# Autodesk Inventor assembly: HbthumbU02
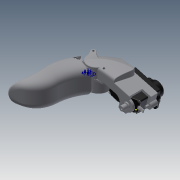
[picture p0: Inventor's stored thumbnail of the model, 180x180]
Saved by Autodesk Inventor 2015 SP1 (Build 190203100, 203)
## iProperties
Created: 2015-02-19
Part Number: HbthumbU02
Document SubType Name: Assembly
Designer: Yamaura
Author: Yamaura
## Documents named in this file (11)
- C:\Users\Yamaura\Documents\GitHub\HACKberry\HACKberry-hardware\3D\Inventor\Parts\HbthumbU02.iam
- C:\Users\Yamaura\Documents\GitHub\HACKberry\HACKberry-hardware\3D\Inventor\Parts\ASV-15MG.ipt
- C:\Users\Yamaura\Documents\GitHub\HACKberry\HACKberry-hardware\3D\Inventor\Parts\HbThumbLockButton01.ipt
- C:\Users\Yamaura\Documents\GitHub\HACKberry\HACKberry-hardware\3D\Inventor\Parts\CP 0.5-6-8.ipt
- C:\Users\Yamaura\Documents\GitHub\HACKberry\HACKberry-hardware\3D\Inventor\Parts\flatScrewM2L6PHI3.3T1.3.ipt
- C:\Users\Yamaura\Documents\GitHub\HACKberry\HACKberry-hardware\3D\Inventor\Parts\ScrewM2L10.ipt
- C:\Users\Yamaura\Documents\GitHub\HACKberry\HACKberry-hardware\3D\Inventor\Parts\HbThumbJointHolder01.ipt
- C:\Users\Yamaura\Documents\GitHub\HACKberry\HACKberry-hardware\3D\Inventor\Parts\HbThumbMetacarpalPhalanx02.ipt
- C:\Users\Yamaura\Documents\GitHub\HACKberry\HACKberry-hardware\3D\Inventor\Parts\HbThumbMetacarpalPhalanxCover02.ipt
- C:\Users\Yamaura\Documents\GitHub\HACKberry\HACKberry-hardware\3D\Inventor\Parts\HbThumbProximalPhalanx02.ipt
- C:\Users\Yamaura\Documents\GitHub\HACKberry\HACKberry-hardware\3D\Inventor\Parts\HbThumbProximalPhalanxBase02.ipt
## Components (11 placed, 10 different names)
1. ASV-15MG:1 — メイト:35, メイト:37, メイト:38, メイト:48, メイト:58
2. ScrewM2L10:1 — メイト:35, メイト:59
3. ScrewM2L10:2 — メイト:37, メイト:38
4. HbThumbLockButton01:1 — メイト:31, 角度:5, メイト:60
5. CP 0.5-6-8:1 — メイト:25
6. flatScrewM2L6PHI3.3T1.3:1
7. HbThumbJointHolder01:1 — メイト:49, メイト:50, メイト:51, 角度:6
8. HbThumbMetacarpalPhalanx02:1 — メイト:47, メイト:48, メイト:50, メイト:51, メイト:56, メイト:57, メイト:60
9. HbThumbMetacarpalPhalanxCover02:1 — メイト:56, メイト:57, メイト:58, メイト:59
10. HbThumbProximalPhalanx02:1 — メイト:54, メイト:55, 角度:7
11. HbThumbProximalPhalanxBase02:1 — メイト:52, メイト:53, 角度:6, メイト:54, メイト:55, 角度:7
## Relationships (23: Mate 20, Angle 3)
- メイト:25 [Mate]: CP 0.5-6-8:1
- メイト:31 [Mate]: HbThumbLockButton01:1
- 角度:5 [Angle] (40 deg): HbThumbLockButton01:1
- メイト:35 [Mate]: ASV-15MG:1 ↔ ScrewM2L10:1
- メイト:37 [Mate]: ASV-15MG:1 ↔ ScrewM2L10:2
- メイト:38 [Mate]: ASV-15MG:1 ↔ ScrewM2L10:2
- メイト:46 [Mate]
- メイト:47 [Mate]: HbThumbMetacarpalPhalanx02:1
- メイト:48 [Mate]: ASV-15MG:1 ↔ HbThumbMetacarpalPhalanx02:1
- メイト:49 [Mate]: HbThumbJointHolder01:1
- メイト:50 [Mate]: HbThumbJointHolder01:1 ↔ HbThumbMetacarpalPhalanx02:1
- メイト:51 [Mate]: HbThumbJointHolder01:1 ↔ HbThumbMetacarpalPhalanx02:1
- メイト:52 [Mate]: HbThumbProximalPhalanxBase02:1
- メイト:53 [Mate] (-1.5 mm): HbThumbProximalPhalanxBase02:1
- 角度:6 [Angle] (180 deg): HbThumbJointHolder01:1 ↔ HbThumbProximalPhalanxBase02:1
- メイト:54 [Mate] (0.2 mm): HbThumbProximalPhalanx02:1 ↔ HbThumbProximalPhalanxBase02:1
- メイト:55 [Mate]: HbThumbProximalPhalanx02:1 ↔ HbThumbProximalPhalanxBase02:1
- 角度:7 [Angle] (180 deg): HbThumbProximalPhalanx02:1 ↔ HbThumbProximalPhalanxBase02:1
- メイト:56 [Mate]: HbThumbMetacarpalPhalanx02:1 ↔ HbThumbMetacarpalPhalanxCover02:1
- メイト:57 [Mate]: HbThumbMetacarpalPhalanx02:1 ↔ HbThumbMetacarpalPhalanxCover02:1
- メイト:58 [Mate]: ASV-15MG:1 ↔ HbThumbMetacarpalPhalanxCover02:1
- メイト:59 [Mate]: ScrewM2L10:1 ↔ HbThumbMetacarpalPhalanxCover02:1
- メイト:60 [Mate]: HbThumbLockButton01:1 ↔ HbThumbMetacarpalPhalanx02:1
